# Autodesk Inventor assembly: 組合1
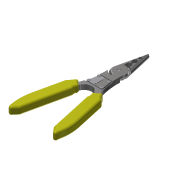
[picture p0: Inventor's stored thumbnail of the model, 180x180]
Saved by Autodesk Inventor 2019 (Build 230136000, 136)
## iProperties
Created: 2022-10-02
Part Number: 組合1
Document SubType Name: Assembly
Designer: user
Author: user
## Documents named in this file (3)
- C:\Users\user\Desktop\組合1.iam
- C:\Users\user\Desktop\零件2.ipt
- C:\Users\user\Desktop\零件3.ipt
## Components (5 placed, 2 different names)
1. 零件2:1 — 貼合:1, 貼合:2, 貼合:3, 貼合:4, 貼合:5, 貼合:6, 貼合:7, 貼合:8
2. 零件3:1 — 貼合:1, 貼合:2
3. 零件3:2 — 貼合:3, 貼合:6
4. 零件3:3 — 貼合:4, 貼合:8
5. 零件3:4 — 貼合:5, 貼合:7
## Relationships (8: Mate 8)
- 貼合:1 [Mate]: 零件2:1 ↔ 零件3:1
- 貼合:2 [Mate]: 零件2:1 ↔ 零件3:1
- 貼合:3 [Mate]: 零件2:1 ↔ 零件3:2
- 貼合:4 [Mate]: 零件2:1 ↔ 零件3:3
- 貼合:5 [Mate]: 零件2:1 ↔ 零件3:4
- 貼合:6 [Mate]: 零件2:1 ↔ 零件3:2
- 貼合:7 [Mate]: 零件2:1 ↔ 零件3:4
- 貼合:8 [Mate]: 零件2:1 ↔ 零件3:3
